# Autodesk Inventor assembly: INDX_000_Main
(part 2 of 2)
- Mate:232: INDX_009_FrontHex:1 ↔ COTS_0.25-20_ButtonHead_0.5inlong_StainlessSteel_92949A537:5
- Mate:233: COTS_90107A029_316 Stainless Steel Washer:3 ↔ COTS_0.25-20_ButtonHead_0.5inlong_StainlessSteel_92949A537:5
- Mate:234: INDX_010_5inHex:1 ↔ COTS_0.25-20_ButtonHead_0.5inlong_StainlessSteel_92949A537:8
- Mate:235: COTS_90107A029_316 Stainless Steel Washer:5 ↔ COTS_0.25-20_ButtonHead_0.5inlong_StainlessSteel_92949A537:8
- Mate:236: INDX_012_OuterPlate:1 ↔ COTS_91251A540_Black-Oxide Alloy Steel Socket Head Screw:2
- Mate:237: INDX_012_OuterPlate:1 ↔ COTS_91251A540_Black-Oxide Alloy Steel Socket Head Screw:2
- Mate:238: INDX_012_OuterPlate:1 ↔ COTS_91251A540_Black-Oxide Alloy Steel Socket Head Screw:1
- Mate:239: INDX_012_OuterPlate:1 ↔ COTS_91251A540_Black-Oxide Alloy Steel Socket Head Screw:1
- Mate:240: INDX_017_Mainhex:3 ↔ COTS_0.25-20_ButtonHead_0.5inlong_StainlessSteel_92949A537:7
- Mate:241: COTS_90107A029_316 Stainless Steel Washer:9 ↔ COTS_0.25-20_ButtonHead_0.5inlong_StainlessSteel_92949A537:7
- Mate:242: COTS_WCP-0783_1.125ODHexBearing:13 ↔ INDX_017_Mainhex:10
- Flush:16: COTS_WCP-0783_1.125ODHexBearing:13 ↔ INDX_017_Mainhex:10
- Mate:243: INDX_011_SecondPlate:1 ↔ COTS_0.25-20_ButtonHead_0.5inlong_StainlessSteel_92949A537:9
- Mate:244: INDX_011_SecondPlate:1 ↔ COTS_0.25-20_ButtonHead_0.5inlong_StainlessSteel_92949A537:9
- Mate:245: INDX_011_SecondPlate:1 ↔ COTS_0.25-20_ButtonHead_0.5inlong_StainlessSteel_92949A537:10
- Mate:246: INDX_011_SecondPlate:1 ↔ COTS_0.25-20_ButtonHead_0.5inlong_StainlessSteel_92949A537:10
- Mate:247: INDX_007_22TPulley:2 ↔ INDX_022_SideBelt:1
- Mate:248: INDX_007_22TPulley:1 ↔ INDX_022_SideBelt:1
- Mate:249 (0.5 mm): INDX_007_22TPulley:1 ↔ INDX_022_SideBelt:1
- Mate:250: COTS_WCP-0783_1.125ODHexBearing:20 ↔ COTS_am-3462_2indiameter_0.500inhexbore_durometer35A_CompliantWheel:11
- Mate:251: COTS_am-3462_2indiameter_0.500inhexbore_durometer35A_CompliantWheel:11 ↔ COTS_am-3462_2indiameter_0.500inhexbore_durometer35A_CompliantWheel:12
- Mate:252: COTS_am-3462_2indiameter_0.500inhexbore_durometer35A_CompliantWheel:9 ↔ COTS_am-3462_2indiameter_0.500inhexbore_durometer35A_CompliantWheel:12
- Mate:253: COTS_am-3462_2indiameter_0.500inhexbore_durometer35A_CompliantWheel:9 ↔ COTS_am-3462_2indiameter_0.500inhexbore_durometer35A_CompliantWheel:10
- Mate:254: COTS_WCP-0783_1.125ODHexBearing:21 ↔ COTS_am-3462_2indiameter_0.500inhexbore_durometer35A_CompliantWheel:15
- Mate:255: COTS_am-3462_2indiameter_0.500inhexbore_durometer35A_CompliantWheel:13 ↔ COTS_am-3462_2indiameter_0.500inhexbore_durometer35A_CompliantWheel:15
- Mate:256: COTS_am-3462_2indiameter_0.500inhexbore_durometer35A_CompliantWheel:14 ↔ COTS_am-3462_2indiameter_0.500inhexbore_durometer35A_CompliantWheel:15
- Mate:257: COTS_am-3462_2indiameter_0.500inhexbore_durometer35A_CompliantWheel:14 ↔ COTS_am-3462_2indiameter_0.500inhexbore_durometer35A_CompliantWheel:16
- Mate:258: COTS_WCP-0783_1.125ODHexBearing:21 ↔ COTS_90107A029_316 Stainless Steel Washer:11
- Mate:259: INDX_017_Mainhex:9 ↔ COTS_90107A029_316 Stainless Steel Washer:11
- Mate:260: COTS_WCP-0783_1.125ODHexBearing:20 ↔ COTS_90107A029_316 Stainless Steel Washer:12
- Mate:261: COTS_WCP-0783_1.125ODHexBearing:20 ↔ COTS_90107A029_316 Stainless Steel Washer:12
- Mate:262: COTS_WCP-0783_1.125ODHexBearing:4 ↔ COTS_90107A029_316 Stainless Steel Washer:14
- Mate:263: COTS_WCP-0783_1.125ODHexBearing:4 ↔ COTS_90107A029_316 Stainless Steel Washer:14
- Mate:264: COTS_WCP-0783_1.125ODHexBearing:1 ↔ COTS_90107A029_316 Stainless Steel Washer:13
- Mate:265: COTS_WCP-0783_1.125ODHexBearing:1 ↔ COTS_90107A029_316 Stainless Steel Washer:13
- Mate:266: COTS_0.25-20_ButtonHead_0.5inlong_StainlessSteel_92949A537:11 ↔ COTS_90107A029_316 Stainless Steel Washer:14
- Mate:267: COTS_0.25-20_ButtonHead_0.5inlong_StainlessSteel_92949A537:11 ↔ COTS_90107A029_316 Stainless Steel Washer:14
- Mate:268: COTS_90107A029_316 Stainless Steel Washer:13 ↔ COTS_0.25-20_ButtonHead_0.5inlong_StainlessSteel_92949A537:14
- Mate:269: COTS_90107A029_316 Stainless Steel Washer:13 ↔ COTS_0.25-20_ButtonHead_0.5inlong_StainlessSteel_92949A537:14
- Mate:270: INDX_017_Mainhex:7 ↔ COTS_0.25-20_ButtonHead_0.5inlong_StainlessSteel_92949A537:12
- Mate:271: COTS_90107A029_316 Stainless Steel Washer:12 ↔ COTS_0.25-20_ButtonHead_0.5inlong_StainlessSteel_92949A537:12
- Mate:272: INDX_017_Mainhex:9 ↔ COTS_0.25-20_ButtonHead_0.5inlong_StainlessSteel_92949A537:13
- Mate:273: COTS_90107A029_316 Stainless Steel Washer:11 ↔ COTS_0.25-20_ButtonHead_0.5inlong_StainlessSteel_92949A537:13
- Mate:274: INDX_002_Standoff:1 ↔ COTS_91251A540_Black-Oxide Alloy Steel Socket Head Screw:3
- Mate:275: INDX_002_Standoff:2 ↔ COTS_91251A540_Black-Oxide Alloy Steel Socket Head Screw:4
- Mate:276: INDX_011_SecondPlate:1 ↔ COTS_91251A540_Black-Oxide Alloy Steel Socket Head Screw:4
- Mate:277: INDX_011_SecondPlate:1 ↔ COTS_91251A540_Black-Oxide Alloy Steel Socket Head Screw:3
- Mate:278: INDX_001_Plate:2 ↔ COTS_91251A540_Black-Oxide Alloy Steel Socket Head Screw:6
- Mate:279: INDX_001_Plate:2 ↔ COTS_91251A540_Black-Oxide Alloy Steel Socket Head Screw:6
- Mate:280: INDX_001_Plate:2 ↔ COTS_91251A540_Black-Oxide Alloy Steel Socket Head Screw:5
- Mate:281: INDX_001_Plate:2 ↔ COTS_91251A540_Black-Oxide Alloy Steel Socket Head Screw:5
- Mate:282: INDX_017_Mainhex:6 ↔ COTS_0.25-20_ButtonHead_0.5inlong_StainlessSteel_92949A537:15
- Mate:283: COTS_90107A029_316 Stainless Steel Washer:8 ↔ COTS_0.25-20_ButtonHead_0.5inlong_StainlessSteel_92949A537:15
- Mate:284: INDX_017_Mainhex:4 ↔ COTS_0.25-20_ButtonHead_0.5inlong_StainlessSteel_92949A537:16
- Mate:285: COTS_90107A029_316 Stainless Steel Washer:7 ↔ COTS_0.25-20_ButtonHead_0.5inlong_StainlessSteel_92949A537:16
- Mate:286: COTS_WCP-0783_1.125ODHexBearing:19 ↔ COTS_90107A029_316 Stainless Steel Washer:16
- Mate:287: INDX_017_Mainhex:8 ↔ COTS_90107A029_316 Stainless Steel Washer:16
- Mate:288: COTS_WCP-0783_1.125ODHexBearing:13 ↔ COTS_90107A029_316 Stainless Steel Washer:15
- Mate:289: INDX_017_Mainhex:10 ↔ COTS_90107A029_316 Stainless Steel Washer:15
- Mate:290: INDX_017_Mainhex:10 ↔ COTS_0.25-20_ButtonHead_0.5inlong_StainlessSteel_92949A537:17
- Mate:291: COTS_90107A029_316 Stainless Steel Washer:15 ↔ COTS_0.25-20_ButtonHead_0.5inlong_StainlessSteel_92949A537:17
- Mate:292: INDX_017_Mainhex:8 ↔ COTS_0.25-20_ButtonHead_0.5inlong_StainlessSteel_92949A537:18
- Mate:293: COTS_90107A029_316 Stainless Steel Washer:16 ↔ COTS_0.25-20_ButtonHead_0.5inlong_StainlessSteel_92949A537:18
- Mate:294: INDX_011_SecondPlate:1 ↔ COTS_91251A540_Black-Oxide Alloy Steel Socket Head Screw:7
- Mate:295: INDX_001_Plate:2 ↔ COTS_91251A540_Black-Oxide Alloy Steel Socket Head Screw:8
- Mate:296: INDX_001_Plate:2 ↔ COTS_91251A540_Black-Oxide Alloy Steel Socket Head Screw:8
- Mate:297: INDX_011_SecondPlate:1 ↔ COTS_91251A540_Black-Oxide Alloy Steel Socket Head Screw:7
- Mate:298: INDX_011_SecondPlate:1 ↔ COTS_91251A540_Black-Oxide Alloy Steel Socket Head Screw:9
- Mate:299: INDX_011_SecondPlate:1 ↔ COTS_91251A540_Black-Oxide Alloy Steel Socket Head Screw:9
- Mate:300: INDX_001_Plate:2 ↔ COTS_91251A540_Black-Oxide Alloy Steel Socket Head Screw:10
- Mate:301: INDX_001_Plate:2 ↔ COTS_91251A540_Black-Oxide Alloy Steel Socket Head Screw:10
- Mate:302: COTS_WCP-0783_1.125ODHexBearing:14 ↔ COTS_HTD5MM_9mm_16TPulley:3
- Mate:303: COTS_WCP-0783_1.125ODHexBearing:17 ↔ COTS_HTD5MM_9mm_16TPulley:4
- Flush:17: COTS_HTD5MM_9mm_16TPulley:3 ↔ COTS_HTD5MM_9mm_16TPulley:4
- Mate:304: COTS_WCP-0783_1.125ODHexBearing:17 ↔ COTS_HTD5MM_9mm_16TPulley:5
- Flush:18: COTS_HTD5MM_9mm_16TPulley:5 ↔ COTS_HTD5MM_9mm_16TPulley:6
- Mate:305: COTS_WCP-0783_1.125ODHexBearing:16 ↔ COTS_HTD5MM_9mm_16TPulley:6
- Mate:306: COTS_WCP-0783_1.125ODHexBearing:6 ↔ COTS_HTD5MM_9mm_16TPulley:7
- Mate:307: COTS_WCP-0783_1.125ODHexBearing:5 ↔ COTS_HTD5MM_9mm_16TPulley:8
- Flush:19: COTS_HTD5MM_9mm_16TPulley:7 ↔ COTS_HTD5MM_9mm_16TPulley:8
- Mate:308: COTS_WCP-0783_1.125ODHexBearing:11 ↔ COTS_HTD5MM_9mm_16TPulley:9
- Mate:309: COTS_WCP-0783_1.125ODHexBearing:19 ↔ COTS_HTD5MM_9mm_16TPulley:10
- Flush:20: COTS_HTD5MM_9mm_16TPulley:9 ↔ COTS_HTD5MM_9mm_16TPulley:10
- Mate:310: COTS_WCP-0783_1.125ODHexBearing:2 ↔ COTS_HTD5MM_9mm_16TPulley:12
- Mate:311: COTS_WCP-0783_1.125ODHexBearing:1 ↔ COTS_HTD5MM_9mm_16TPulley:11
- Flush:21: COTS_HTD5MM_9mm_16TPulley:11 ↔ COTS_HTD5MM_9mm_16TPulley:12
- Mate:312: COTS_WCP-0783_1.125ODHexBearing:26 ↔ COTS_HTD5MM_9mm_16TPulley:14
- Mate:313: COTS_WCP-0783_1.125ODHexBearing:12 ↔ COTS_HTD5MM_9mm_16TPulley:13
- Mate:314: COTS_WCP-0783_1.125ODHexBearing:15 ↔ COTS_HTD5MM_9mm_16TPulley:15
- Mate:315: COTS_WCP-0783_1.125ODHexBearing:15 ↔ COTS_HTD5MM_9mm_16TPulley:16
- Flush:22: COTS_HTD5MM_9mm_16TPulley:14 ↔ COTS_HTD5MM_9mm_16TPulley:16
- Flush:23: COTS_HTD5MM_9mm_16TPulley:13 ↔ COTS_HTD5MM_9mm_16TPulley:15
- Mate:316: COTS_WCP-0783_1.125ODHexBearing:12 ↔ COTS_HTD5MM_9mm_16TPulley:19
- Mate:317: COTS_WCP-0783_1.125ODHexBearing:13 ↔ COTS_HTD5MM_9mm_16TPulley:20
- Flush:24: COTS_HTD5MM_9mm_16TPulley:19 ↔ COTS_HTD5MM_9mm_16TPulley:20
- Mate:318: COTS_WCP-0783_1.125ODHexBearing:3 ↔ COTS_HTD5MM_9mm_16TPulley:17
- Mate:319: COTS_WCP-0783_1.125ODHexBearing:4 ↔ COTS_HTD5MM_9mm_16TPulley:18
- Flush:25: COTS_HTD5MM_9mm_16TPulley:17 ↔ COTS_HTD5MM_9mm_16TPulley:18
- Mate:320: COTS_WCP-0783_1.125ODHexBearing:27 ↔ COTS_90107A029_316 Stainless Steel Washer:17
- Mate:321: INDX_015_OuterHex:1 ↔ COTS_90107A029_316 Stainless Steel Washer:17
- Mate:322: INDX_015_OuterHex:1 ↔ COTS_0.25-20_ButtonHead_0.5inlong_StainlessSteel_92949A537:19
- Mate:323: COTS_90107A029_316 Stainless Steel Washer:17 ↔ COTS_0.25-20_ButtonHead_0.5inlong_StainlessSteel_92949A537:19
- Mate:324: COTS_HTD5MM_9mm_16TPulley:14 ↔ INDX_023_MainBelt:3
- Mate:325: COTS_HTD5MM_9mm_16TPulley:16 ↔ INDX_023_MainBelt:3
- Mate:326 (1 mm): COTS_HTD5MM_9mm_16TPulley:16 ↔ INDX_023_MainBelt:3
- Mate:327: COTS_HTD5MM_9mm_16TPulley:15 ↔ INDX_023_MainBelt:2
- Mate:328: COTS_HTD5MM_9mm_16TPulley:13 ↔ INDX_023_MainBelt:2
- Mate:329 (1.5 mm): COTS_HTD5MM_9mm_16TPulley:15 ↔ INDX_023_MainBelt:2
- Mate:330: COTS_HTD5MM_9mm_16TPulley:19 ↔ INDX_023_MainBelt:1
- Mate:331: COTS_HTD5MM_9mm_16TPulley:20 ↔ INDX_023_MainBelt:1
- Mate:332 (1.5 mm): COTS_HTD5MM_9mm_16TPulley:20 ↔ INDX_023_MainBelt:1
- Mate:333: COTS_HTD5MM_9mm_16TPulley:17 ↔ INDX_023_MainBelt:4
- Mate:334: COTS_HTD5MM_9mm_16TPulley:18 ↔ INDX_023_MainBelt:4
- Mate:335 (1.5 mm): COTS_HTD5MM_9mm_16TPulley:17 ↔ INDX_023_MainBelt:4
- Mate:336: COTS_HTD5MM_9mm_16TPulley:3 ↔ INDX_023_MainBelt:9
- Mate:337: COTS_HTD5MM_9mm_16TPulley:4 ↔ INDX_023_MainBelt:9
- Mate:338 (1.5 mm): COTS_HTD5MM_9mm_16TPulley:4 ↔ INDX_023_MainBelt:9
- Mate:339: COTS_HTD5MM_9mm_16TPulley:5 ↔ INDX_023_MainBelt:8
- Mate:340: COTS_HTD5MM_9mm_16TPulley:6 ↔ INDX_023_MainBelt:8
- Mate:341 (1.5 mm): COTS_HTD5MM_9mm_16TPulley:6 ↔ INDX_023_MainBelt:8
- Mate:342: COTS_HTD5MM_9mm_16TPulley:9 ↔ INDX_023_MainBelt:6
- Mate:343 (1.5 mm): COTS_HTD5MM_9mm_16TPulley:9 ↔ INDX_023_MainBelt:6
- Mate:344: COTS_HTD5MM_9mm_16TPulley:10 ↔ INDX_023_MainBelt:6
- Mate:345: COTS_HTD5MM_9mm_16TPulley:7 ↔ INDX_023_MainBelt:5
- Mate:346: COTS_HTD5MM_9mm_16TPulley:8 ↔ INDX_023_MainBelt:5
- Mate:347 (1.5 mm): COTS_HTD5MM_9mm_16TPulley:8 ↔ INDX_023_MainBelt:5
- Mate:348: COTS_HTD5MM_9mm_16TPulley:12 ↔ INDX_023_MainBelt:7
- Mate:349: COTS_HTD5MM_9mm_16TPulley:11 ↔ INDX_023_MainBelt:7
- Mate:350 (1.5 mm): COTS_HTD5MM_9mm_16TPulley:11 ↔ INDX_023_MainBelt:7
- Mate:351: INDX_001_Plate:2 ↔ COTS_91251A540_Black-Oxide Alloy Steel Socket Head Screw:11
- Mate:352: INDX_001_Plate:2 ↔ COTS_91251A540_Black-Oxide Alloy Steel Socket Head Screw:11
- Mate:353: INDX_001_Plate:2 ↔ COTS_91251A540_Black-Oxide Alloy Steel Socket Head Screw:11
- Mate:354: COTS_WCP-0783_1.125ODHexBearing:10 ↔ COTS_90107A029_316 Stainless Steel Washer:19
- Mate:355: INDX_017_Mainhex:2 ↔ COTS_90107A029_316 Stainless Steel Washer:19
- Mate:356: COTS_WCP-0783_1.125ODHexBearing:8 ↔ COTS_90107A029_316 Stainless Steel Washer:18
- Mate:357: INDX_017_Mainhex:1 ↔ COTS_90107A029_316 Stainless Steel Washer:18
- Mate:358: COTS_WCP-0783_1.125ODHexBearing:7 ↔ COTS_90107A029_316 Stainless Steel Washer:20
- Mate:359: INDX_017_Mainhex:5 ↔ COTS_90107A029_316 Stainless Steel Washer:20
- Mate:360: INDX_001_Plate:2 ↔ COTS_91251A540_Black-Oxide Alloy Steel Socket Head Screw:12
- Mate:361: INDX_001_Plate:2 ↔ COTS_91251A540_Black-Oxide Alloy Steel Socket Head Screw:12
- Mate:362: COTS_WCP-0783_1.125ODHexBearing:6 ↔ COTS_90107A029_316 Stainless Steel Washer:21
- Mate:363: INDX_017_Mainhex:4 ↔ COTS_90107A029_316 Stainless Steel Washer:21
- Mate:364: COTS_WCP-0783_1.125ODHexBearing:5 ↔ COTS_90107A029_316 Stainless Steel Washer:22
- Mate:365: INDX_017_Mainhex:6 ↔ COTS_90107A029_316 Stainless Steel Washer:22
- Mate:366: COTS_WCP-0783_1.125ODHexBearing:9 ↔ COTS_90107A029_316 Stainless Steel Washer:23
- Mate:367: INDX_017_Mainhex:3 ↔ COTS_90107A029_316 Stainless Steel Washer:23
- Mate:368: COTS_WCP-0783_1.125ODHexBearing:3 ↔ COTS_90107A029_316 Stainless Steel Washer:25
- Mate:369: INDX_017_Mainhex:10 ↔ COTS_90107A029_316 Stainless Steel Washer:25
- Mate:370: COTS_WCP-0783_1.125ODHexBearing:2 ↔ COTS_90107A029_316 Stainless Steel Washer:24
- Mate:371: INDX_017_Mainhex:8 ↔ COTS_90107A029_316 Stainless Steel Washer:24
- Mate:372: INDX_017_Mainhex:10 ↔ COTS_0.25-20_ButtonHead_0.5inlong_StainlessSteel_92949A537:20
- Mate:373: INDX_017_Mainhex:8 ↔ COTS_0.25-20_ButtonHead_0.5inlong_StainlessSteel_92949A537:21
- Mate:374: COTS_90107A029_316 Stainless Steel Washer:24 ↔ COTS_0.25-20_ButtonHead_0.5inlong_StainlessSteel_92949A537:21
- Mate:375: COTS_90107A029_316 Stainless Steel Washer:25 ↔ COTS_0.25-20_ButtonHead_0.5inlong_StainlessSteel_92949A537:20
- Mate:376: COTS_WCP-0783_1.125ODHexBearing:24 ↔ COTS_90107A029_316 Stainless Steel Washer:26
- Mate:377: INDX_016_BottomHex:1 ↔ COTS_90107A029_316 Stainless Steel Washer:26
- Mate:378: INDX_016_BottomHex:1 ↔ COTS_0.25-20_ButtonHead_0.5inlong_StainlessSteel_92949A537:23
- Mate:379: COTS_0.25-20_ButtonHead_0.5inlong_StainlessSteel_92949A537:23 ↔ COTS_90107A029_316 Stainless Steel Washer:26
- Mate:380: INDX_017_Mainhex:2 ↔ COTS_0.25-20_ButtonHead_0.5inlong_StainlessSteel_92949A537:25
- Mate:381: COTS_90107A029_316 Stainless Steel Washer:19 ↔ COTS_0.25-20_ButtonHead_0.5inlong_StainlessSteel_92949A537:25
- Mate:382: INDX_017_Mainhex:1 ↔ COTS_0.25-20_ButtonHead_0.5inlong_StainlessSteel_92949A537:24
- Mate:383: COTS_90107A029_316 Stainless Steel Washer:18 ↔ COTS_0.25-20_ButtonHead_0.5inlong_StainlessSteel_92949A537:24
- Mate:384: INDX_017_Mainhex:4 ↔ COTS_0.25-20_ButtonHead_0.5inlong_StainlessSteel_92949A537:22
- Mate:385: COTS_90107A029_316 Stainless Steel Washer:21 ↔ COTS_0.25-20_ButtonHead_0.5inlong_StainlessSteel_92949A537:22
- Mate:386: INDX_017_Mainhex:5 ↔ COTS_0.25-20_ButtonHead_0.5inlong_StainlessSteel_92949A537:26
- Mate:387: COTS_90107A029_316 Stainless Steel Washer:20 ↔ COTS_0.25-20_ButtonHead_0.5inlong_StainlessSteel_92949A537:26
- Mate:389: INDX_001_Plate:2 ↔ COTS_91860A047_Size10Washer:1
- Mate:390: INDX_001_Plate:2 ↔ COTS_91860A047_Size10Washer:1
- Mate:391: COTS_91860A047_Size10Washer:1 ↔ COTS_91251A350_7-16in Long_Black-Oxide Alloy Steel Socket Head:1
- Mate:392: COTS_91860A047_Size10Washer:1 ↔ COTS_91251A350_7-16in Long_Black-Oxide Alloy Steel Socket Head:1
- Mate:393: INDX_001_Plate:2 ↔ COTS_91860A047_Size10Washer:4
- Mate:394: INDX_001_Plate:2 ↔ COTS_91860A047_Size10Washer:2
- Mate:395: INDX_001_Plate:2 ↔ COTS_91860A047_Size10Washer:3
- Mate:396: INDX_001_Plate:2 ↔ COTS_91860A047_Size10Washer:4
- Mate:397: INDX_001_Plate:2 ↔ COTS_91860A047_Size10Washer:2
- Mate:398: INDX_001_Plate:2 ↔ COTS_91860A047_Size10Washer:3
- Mate:399: INDX_001_Plate:2 ↔ COTS_91251A350_7-16in Long_Black-Oxide Alloy Steel Socket Head:2
- Mate:400: INDX_001_Plate:2 ↔ COTS_91251A350_7-16in Long_Black-Oxide Alloy Steel Socket Head:3
- Mate:401: INDX_001_Plate:2 ↔ COTS_91251A350_7-16in Long_Black-Oxide Alloy Steel Socket Head:4
- Mate:402: COTS_91860A047_Size10Washer:2 ↔ COTS_91251A350_7-16in Long_Black-Oxide Alloy Steel Socket Head:3
- Mate:403: COTS_91860A047_Size10Washer:3 ↔ COTS_91251A350_7-16in Long_Black-Oxide Alloy Steel Socket Head:4
- Mate:404: COTS_WCP-0783_1.125ODHexBearing:14 ↔ COTS_am-3462_2indiameter_0.500inhexbore_durometer60A_CompliantWheel:2
- Mate:405: COTS_WCP-0783_1.125ODHexBearing:14 ↔ COTS_am-3462_2indiameter_0.500inhexbore_durometer60A_CompliantWheel:1
- Mate:406: COTS_am-3462_2indiameter_0.500inhexbore_durometer60A_CompliantWheel:1 ↔ COTS_am-3462_2indiameter_0.500inhexbore_durometer60A_CompliantWheel:3
- Mate:407: COTS_am-3462_2indiameter_0.500inhexbore_durometer60A_CompliantWheel:3 ↔ COTS_am-3462_2indiameter_0.500inhexbore_durometer60A_CompliantWheel:4
- Mate:408: COTS_WCP-0783_1.125ODHexBearing:15 ↔ COTS_am-3462_2indiameter_0.500inhexbore_durometer60A_CompliantWheel:5
- Mate:409: COTS_am-3462_2indiameter_0.500inhexbore_durometer60A_CompliantWheel:5 ↔ COTS_am-3462_2indiameter_0.500inhexbore_durometer60A_CompliantWheel:7
- Mate:410: COTS_am-3462_2indiameter_0.500inhexbore_durometer60A_CompliantWheel:6 ↔ COTS_am-3462_2indiameter_0.500inhexbore_durometer60A_CompliantWheel:7
- Mate:411: COTS_am-3462_2indiameter_0.500inhexbore_durometer60A_CompliantWheel:6 ↔ COTS_am-3462_2indiameter_0.500inhexbore_durometer60A_CompliantWheel:8
- Mate:412: COTS_WCP-0783_1.125ODHexBearing:17 ↔ COTS_am-3462_2indiameter_0.500inhexbore_durometer60A_CompliantWheel:9
- Mate:413: COTS_am-3462_2indiameter_0.500inhexbore_durometer60A_CompliantWheel:9 ↔ COTS_am-3462_2indiameter_0.500inhexbore_durometer60A_CompliantWheel:10
- Mate:414: COTS_am-3462_2indiameter_0.500inhexbore_durometer60A_CompliantWheel:9 ↔ COTS_am-3462_2indiameter_0.500inhexbore_durometer60A_CompliantWheel:11
- Mate:415: COTS_am-3462_2indiameter_0.500inhexbore_durometer60A_CompliantWheel:11 ↔ COTS_am-3462_2indiameter_0.500inhexbore_durometer60A_CompliantWheel:12
- Mate:416: COTS_WCP-0783_1.125ODHexBearing:16 ↔ COTS_am-3462_2indiameter_0.500inhexbore_durometer60A_CompliantWheel:14
- Mate:417: COTS_am-3462_2indiameter_0.500inhexbore_durometer60A_CompliantWheel:13 ↔ COTS_am-3462_2indiameter_0.500inhexbore_durometer60A_CompliantWheel:14
- Mate:418: COTS_am-3462_2indiameter_0.500inhexbore_durometer60A_CompliantWheel:14 ↔ COTS_am-3462_2indiameter_0.500inhexbore_durometer60A_CompliantWheel:15
- Mate:419: COTS_am-3462_2indiameter_0.500inhexbore_durometer60A_CompliantWheel:15 ↔ COTS_am-3462_2indiameter_0.500inhexbore_durometer60A_CompliantWheel:16
- Mate:420: INDX_011_SecondPlate:1 ↔ COTS_0.25-20_ButtonHead_0.5inlong_StainlessSteel_92949A537:27
- Mate:421: INDX_011_SecondPlate:1 ↔ COTS_0.25-20_ButtonHead_0.5inlong_StainlessSteel_92949A537:28
- Mate:422: INDX_011_SecondPlate:1 ↔ COTS_0.25-20_ButtonHead_0.5inlong_StainlessSteel_92949A537:27
- Mate:423: INDX_011_SecondPlate:1 ↔ COTS_0.25-20_ButtonHead_0.5inlong_StainlessSteel_92949A537:28
- Mate:424: INDX_006_Funnel:2 ↔ COTS_90631A411_10-32_Nylock_Nut:1
- Mate:425: INDX_006_Funnel:2 ↔ COTS_90631A411_10-32_Nylock_Nut:1
- Mate:426: INDX_006_Funnel:2 ↔ COTS_90631A411_10-32_Nylock_Nut:4
- Mate:427: INDX_006_Funnel:2 ↔ COTS_90631A411_10-32_Nylock_Nut:4
- Mate:428: INDX_006_Funnel:2 ↔ COTS_90631A411_10-32_Nylock_Nut:2
- Mate:429: INDX_006_Funnel:2 ↔ COTS_90631A411_10-32_Nylock_Nut:2
- Mate:430: INDX_006_Funnel:2 ↔ COTS_90631A411_10-32_Nylock_Nut:3
- Mate:431: INDX_006_Funnel:2 ↔ COTS_90631A411_10-32_Nylock_Nut:3
- Mate:432: INDX_001_Plate:2 ↔ COTS_0.25-20_ButtonHead_0.5inlong_StainlessSteel_92949A537:29
- Mate:433: INDX_001_Plate:2 ↔ COTS_0.25-20_ButtonHead_0.5inlong_StainlessSteel_92949A537:30
- Mate:434: INDX_001_Plate:2 ↔ COTS_0.25-20_ButtonHead_0.5inlong_StainlessSteel_92949A537:31
- Mate:435: INDX_001_Plate:2 ↔ COTS_0.25-20_ButtonHead_0.5inlong_StainlessSteel_92949A537:32
- Mate:436: INDX_001_Plate:2 ↔ COTS_0.25-20_ButtonHead_0.5inlong_StainlessSteel_92949A537:29
- Mate:437: INDX_001_Plate:2 ↔ COTS_0.25-20_ButtonHead_0.5inlong_StainlessSteel_92949A537:30
- Mate:438: INDX_001_Plate:2 ↔ COTS_0.25-20_ButtonHead_0.5inlong_StainlessSteel_92949A537:32
- Mate:439: INDX_001_Plate:2 ↔ COTS_0.25-20_ButtonHead_0.5inlong_StainlessSteel_92949A537:31
- Mate:440: INDX_006_Funnel:1 ↔ COTS_90631A411_10-32_Nylock_Nut:7
- Mate:441: INDX_006_Funnel:1 ↔ COTS_90631A411_10-32_Nylock_Nut:5
- Mate:442: INDX_006_Funnel:1 ↔ COTS_90631A411_10-32_Nylock_Nut:6
- Mate:443: INDX_006_Funnel:1 ↔ COTS_90631A411_10-32_Nylock_Nut:8
- Mate:444: INDX_006_Funnel:1 ↔ COTS_90631A411_10-32_Nylock_Nut:8
- Mate:446: INDX_006_Funnel:1 ↔ COTS_90631A411_10-32_Nylock_Nut:7
- Mate:447: INDX_006_Funnel:1 ↔ COTS_90631A411_10-32_Nylock_Nut:6
- Mate:448: INDX_006_Funnel:1 ↔ COTS_90631A411_10-32_Nylock_Nut:5
